# Autodesk Inventor assembly: Guntas_Belt_Wheel_Assembly
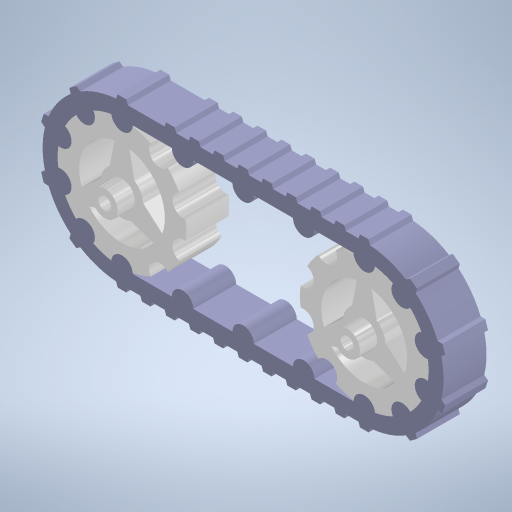
[picture p0: Inventor's stored thumbnail of the model, 512x512]
Saved by Autodesk Inventor 2024 (Build 280153000, 153)
## iProperties
Created: 2023-07-07
Part Number: Guntas_Belt_Wheel_Assembly
Document SubType Name: Assembly
Designer: manas
Author: manas
## Documents named in this file (3)
- C:\Users\manas\Desktop\Guntas_Belt_Wheel_Assembly.iam
- C:\Users\manas\Desktop\Guntas_Belt_New.ipt
- C:\Users\manas\Desktop\Guntas_Wheel_New.ipt
## Components (3 placed, 2 different names)
1. Guntas_Belt_New:1 — Mate:1, Flush:1, Mate:2, Flush:2
2. Guntas_Wheel_New:1 — Mate:1, Flush:1
3. Guntas_Wheel_New:2 — Mate:2, Flush:2
## Relationships (4: Mate 2, Flush 2)
- Mate:1: Guntas_Belt_New:1 ↔ Guntas_Wheel_New:1
- Flush:1: Guntas_Belt_New:1 ↔ Guntas_Wheel_New:1
- Mate:2: Guntas_Belt_New:1 ↔ Guntas_Wheel_New:2
- Flush:2: Guntas_Belt_New:1 ↔ Guntas_Wheel_New:2
